# Autodesk Inventor assembly: 000-base_wheel-v3
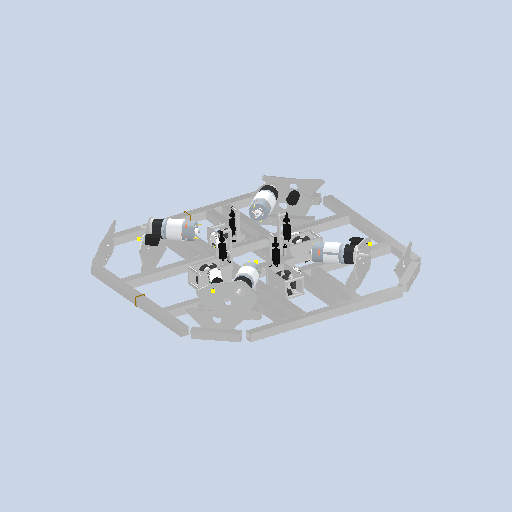
[picture p0: Inventor's stored thumbnail of the model, 512x512]
Saved by Autodesk Inventor 2025.2 (Build 292293000, 293)
## iProperties
Created: 2025-04-01
Part Number: 000-base_wheel-v3
Document SubType Name: Assembly
Designer: haruy
Author: haruy
## Documents named in this file (9)
- C:\Users\haruy\Documents\ロボコン\NHK2025\cad\nagahisa\base_weel\000-base_wheel-v3.iam
- C:\Users\haruy\Documents\ロボコン\NHK2025\cad\nagahisa\base_weel\base_weel-v3-ASP-Base.ipt
- C:\Users\haruy\Documents\ロボコン\NHK2025\cad\nagahisa\base_weel\base_weel-v3-Plate-1.ipt
- C:\Users\haruy\Documents\ロボコン\NHK2025\cad\nagahisa\base_weel\base_weel-v3-Plate-2.ipt
- C:\Users\haruy\Documents\ロボコン\NHK2025\cad\nagahisa\base_weel\takagi_weel\Workspaces\作業スペース\takagi\omuni_wheel_ver3.0\parts\frequently used parts\モーター\RS775\rs775_4.iam
- C:\Users\haruy\Documents\ロボコン\NHK2025\cad\000_parts\エンコーダー\encoder v2.ipt
- C:\Users\haruy\Documents\ロボコン\NHK2025\cad\nagahisa\odom\odom_v1_Plate_5.ipt
- C:\Users\haruy\Documents\ロボコン\NHK2025\cad\nagahisa\odom\000-odom-v1.iam
- C:\Users\haruy\Documents\ロボコン\NHK2025\cad\nagahisa\odom\odom_v1_Plate_6.ipt
## Components (25 placed, 8 different names)
1. base_weel-v3-ASP-Base:1 — 挿入:1, 挿入:2, 挿入:3, 挿入:4, 挿入:5, 挿入:6, 挿入:7, 挿入:8, 挿入:9, 挿入:10, 挿入:11, 挿入:12, 挿入:13, 挿入:14, 挿入:15, 挿入:16, 挿入:25, 挿入:26, 挿入:27, 挿入:28, 挿入:35, 挿入:36, 挿入:37, 挿入:38
2. base_weel-v3-Plate-1:1 — 挿入:1, 挿入:2
3. base_weel-v3-Plate-1:2 — 挿入:3, 挿入:4
4. base_weel-v3-Plate-1:3 — 挿入:7, 挿入:8
5. base_weel-v3-Plate-1:4 — 挿入:5, 挿入:6
6. base_weel-v3-Plate-2:1 — 挿入:9, 挿入:10, 挿入:17, 挿入:23
7. base_weel-v3-Plate-2:2 — 挿入:11, 挿入:12, 挿入:20, 挿入:21
8. base_weel-v3-Plate-2:3 — 挿入:13, 挿入:14, 挿入:18, 挿入:24
9. base_weel-v3-Plate-2:4 — 挿入:15, 挿入:16, 挿入:19, 挿入:22
10. rs775_4:1 [sub-assembly] — 挿入:17
11. rs775_4:2 [sub-assembly] — 挿入:18
12. rs775_4:3 [sub-assembly] — 挿入:19
13. rs775_4:4 [sub-assembly] — 挿入:20
14. encoder v2:1 — 挿入:21
15. encoder v2:2 — 挿入:22
16. encoder v2:3 — 挿入:23
17. encoder v2:4 — 挿入:24
18. odom_v1_Plate_5:1 — 挿入:26, 挿入:28, 挿入:29, 挿入:30, 挿入:31
19. odom_v1_Plate_5:2 — 挿入:25, 挿入:27, 挿入:32, 挿入:33, 挿入:34
20. 000-odom-v1:1 [sub-assembly] — 挿入:29, 挿入:30, 挿入:31
21. 000-odom-v1:2 [sub-assembly] — 挿入:32, 挿入:33, 挿入:34
22. odom_v1_Plate_6:1 — 挿入:35, 挿入:36, 挿入:39, 挿入:40, 挿入:41
23. odom_v1_Plate_6:2 — 挿入:37, 挿入:38, 挿入:42, 挿入:43, 挿入:44
24. 000-odom-v1:3 [sub-assembly] — 挿入:39, 挿入:40, 挿入:41
25. 000-odom-v1:4 [sub-assembly] — 挿入:42, 挿入:43, 挿入:44
## Relationships (44: Insert 44)
- 挿入:1 [Insert]: base_weel-v3-ASP-Base:1 ↔ base_weel-v3-Plate-1:1
- 挿入:2 [Insert]: base_weel-v3-ASP-Base:1 ↔ base_weel-v3-Plate-1:1
- 挿入:3 [Insert]: base_weel-v3-ASP-Base:1 ↔ base_weel-v3-Plate-1:2
- 挿入:4 [Insert]: base_weel-v3-ASP-Base:1 ↔ base_weel-v3-Plate-1:2
- 挿入:5 [Insert]: base_weel-v3-ASP-Base:1 ↔ base_weel-v3-Plate-1:4
- 挿入:6 [Insert]: base_weel-v3-ASP-Base:1 ↔ base_weel-v3-Plate-1:4
- 挿入:7 [Insert]: base_weel-v3-ASP-Base:1 ↔ base_weel-v3-Plate-1:3
- 挿入:8 [Insert]: base_weel-v3-ASP-Base:1 ↔ base_weel-v3-Plate-1:3
- 挿入:9 [Insert]: base_weel-v3-ASP-Base:1 ↔ base_weel-v3-Plate-2:1
- 挿入:10 [Insert]: base_weel-v3-ASP-Base:1 ↔ base_weel-v3-Plate-2:1
- 挿入:11 [Insert]: base_weel-v3-ASP-Base:1 ↔ base_weel-v3-Plate-2:2
- 挿入:12 [Insert]: base_weel-v3-ASP-Base:1 ↔ base_weel-v3-Plate-2:2
- 挿入:13 [Insert]: base_weel-v3-ASP-Base:1 ↔ base_weel-v3-Plate-2:3
- 挿入:14 [Insert]: base_weel-v3-ASP-Base:1 ↔ base_weel-v3-Plate-2:3
- 挿入:15 [Insert]: base_weel-v3-ASP-Base:1 ↔ base_weel-v3-Plate-2:4
- 挿入:16 [Insert]: base_weel-v3-ASP-Base:1 ↔ base_weel-v3-Plate-2:4
- 挿入:17 [Insert]: base_weel-v3-Plate-2:1 ↔ rs775_4:1
- 挿入:18 [Insert]: base_weel-v3-Plate-2:3 ↔ rs775_4:2
- 挿入:19 [Insert]: base_weel-v3-Plate-2:4 ↔ rs775_4:3
- 挿入:20 [Insert]: base_weel-v3-Plate-2:2 ↔ rs775_4:4
- 挿入:21 [Insert]: base_weel-v3-Plate-2:2 ↔ encoder v2:1
- 挿入:22 [Insert]: base_weel-v3-Plate-2:4 ↔ encoder v2:2
- 挿入:23 [Insert]: base_weel-v3-Plate-2:1 ↔ encoder v2:3
- 挿入:24 [Insert]: base_weel-v3-Plate-2:3 ↔ encoder v2:4
- 挿入:25 [Insert]: base_weel-v3-ASP-Base:1 ↔ odom_v1_Plate_5:2
- 挿入:26 [Insert]: base_weel-v3-ASP-Base:1 ↔ odom_v1_Plate_5:1
- 挿入:27 [Insert]: base_weel-v3-ASP-Base:1 ↔ odom_v1_Plate_5:2
- 挿入:28 [Insert]: base_weel-v3-ASP-Base:1 ↔ odom_v1_Plate_5:1
- 挿入:29 [Insert]: odom_v1_Plate_5:1 ↔ 000-odom-v1:1
- 挿入:30 [Insert]: odom_v1_Plate_5:1 ↔ 000-odom-v1:1
- 挿入:31 [Insert]: odom_v1_Plate_5:1 ↔ 000-odom-v1:1
- 挿入:32 [Insert]: odom_v1_Plate_5:2 ↔ 000-odom-v1:2
- 挿入:33 [Insert]: odom_v1_Plate_5:2 ↔ 000-odom-v1:2
- 挿入:34 [Insert]: odom_v1_Plate_5:2 ↔ 000-odom-v1:2
- 挿入:35 [Insert]: base_weel-v3-ASP-Base:1 ↔ odom_v1_Plate_6:1
- 挿入:36 [Insert]: base_weel-v3-ASP-Base:1 ↔ odom_v1_Plate_6:1
- 挿入:37 [Insert]: base_weel-v3-ASP-Base:1 ↔ odom_v1_Plate_6:2
- 挿入:38 [Insert]: base_weel-v3-ASP-Base:1 ↔ odom_v1_Plate_6:2
- 挿入:39 [Insert]: odom_v1_Plate_6:1 ↔ 000-odom-v1:3
- 挿入:40 [Insert]: odom_v1_Plate_6:1 ↔ 000-odom-v1:3
- 挿入:41 [Insert]: odom_v1_Plate_6:1 ↔ 000-odom-v1:3
- 挿入:42 [Insert]: odom_v1_Plate_6:2 ↔ 000-odom-v1:4
- 挿入:43 [Insert]: odom_v1_Plate_6:2 ↔ 000-odom-v1:4
- 挿入:44 [Insert]: odom_v1_Plate_6:2 ↔ 000-odom-v1:4
